# Autodesk Inventor assembly: Servo mount + servo
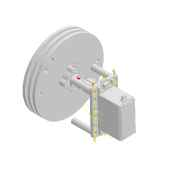
[picture p0: Inventor's stored thumbnail of the model, 180x180]
Saved by Autodesk Inventor 2020 (Build 240168000, 168)
## iProperties
Created: 2020-01-01
Part Number: Servo mount + servo
Document SubType Name: Assembly
Designer: ball
Author: ball
## Documents named in this file (7)
- C:\FTC\FTC8863CAD\2019 Robot\Delivery\extension arm\Servo mount + servo.iam
- C:\FTC\FTC8863CAD\2019 Robot\Delivery\extension arm\whole servo mount.ipt
- C:\FTC\FTC8863CAD\2019 Robot\Delivery\extension arm\servo.iam
- C:\FTC\FTC8863CAD\2019 Robot\Delivery\extension arm\extension arm spool assembly.iam
- C:\FTC\FTC8863CAD\Actobotics\535 parts\535042.ipt
- C:\FTC\FTC8863CAD\2019 Robot\Delivery\extension arm\servo shaft spacer short.ipt
- C:\FTC\FTC8863CAD\2019 Robot\Delivery\extension arm\servo shaft spacer long.ipt
## Components (7 placed, 6 different names)
1. whole servo mount:1 — Mate:3, Mate:4, Mate:5, Mate:6
2. servo:1 [sub-assembly]
3. 535042:1 — Mate:3, Mate:4, Mate:12
4. 535042:2 — Mate:5, Mate:6, Mate:9, Mate:10
5. extension arm spool assembly:2 [sub-assembly] — Mate:7, Mate:8, Mate:11
6. servo shaft spacer short:2 — Mate:7, Mate:8, Mate:9, Mate:10
7. servo shaft spacer long:1 — Mate:11, Mate:12
## Relationships (12: Mate 12)
- [Mate]: whole servo mount:1 ↔ servo:1
- [Mate]: whole servo mount:1 ↔ servo:1
- Mate:3: whole servo mount:1 ↔ 535042:1
- Mate:4: whole servo mount:1 ↔ 535042:1
- Mate:5: whole servo mount:1 ↔ 535042:2
- Mate:6: whole servo mount:1 ↔ 535042:2
- Mate:7: extension arm spool assembly:2 ↔ servo shaft spacer short:2
- Mate:8: extension arm spool assembly:2 ↔ servo shaft spacer short:2
- Mate:9: 535042:2 ↔ servo shaft spacer short:2
- Mate:10: 535042:2 ↔ servo shaft spacer short:2
- Mate:11: extension arm spool assembly:2 ↔ servo shaft spacer long:1
- Mate:12: 535042:1 ↔ servo shaft spacer long:1
